# Autodesk Inventor assembly: RearWheelNoLogo
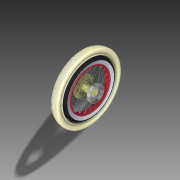
[picture p0: Inventor's stored thumbnail of the model, 180x180]
Saved by Autodesk Inventor 2016 (Build 200138000, 138)
## iProperties
Shininess: 20.0
Length Units: 11269
Angle Units: 11279
Time Units: 11290
Mass Units: 11286
Length Display Precision: 3
Angle Display Precision: 2
Compacted: True
Created: 2001-05-25
Part Number: RearWheelNoLogo
Document SubType Name: Assembly
Designer: Administrator
Density: 0.0
Volumn: 0.0
Area: 0.0
PropertySet Name: Model Information
Control State: 0
Master: False
Checked Out: False
Author: Administrator
## iProperties of the stored document Disk Brake Rotor 230mm.ipt
Created: 2009-08-30
Part Number: Disk Brake Rotor 230mm
Material: SolidWorks Materials|Chrome Stainless Steel|7
Document SubType Name: Modeling
Designer: Yann
Density: 7.8 g/cm^3
Appearance: 229,229,229
Sending System: SolidWorks 2009
Last Author: Administrateur
Last Saved: 2010-11-28
Author: Yann
## Documents named in this file (10)
- **C:\Users\Yann\Documents\GitHub\BIKAIR_CAD\Source\Front_Train\Wheel_spokes\Wheel_spokes.iam*LocalDocs*xCgsrsr1eFgdoe3oxKhlmmklgKg*Disk Brake Rotor 230mm.ipt
- C:\Users\Yann\Documents\GitHub\BIKAIR_CAD\Source\Front_Train\Wheel_spokes\Wheel_spokes.iam
- C:\Users\Yann\Documents\GitHub\BIKAIR_CAD\Source\Front_Train\Wheel_spokes\RearHub.ipt
- C:\Users\Yann\Documents\GitHub\BIKAIR_CAD\Source\Front_Train\Wheel_spokes\ClincherRim2.ipt
- C:\Users\Yann\Documents\GitHub\BIKAIR_CAD\Source\Front_Train\Wheel_spokes\SpokeRear.ipt
- C:\Users\Yann\Documents\GitHub\BIKAIR_CAD\Source\Front_Train\Wheel_spokes\FrontTire.ipt
- C:\Users\Yann\Documents\GitHub\BIKAIR_CAD\Source\Front_Train\Wheel_spokes\RearSprocket.ipt
- C:\Users\Yann\Documents\GitHub\BIKAIR_CAD\Source\Front_Train\Wheel_spokes\BrakeDrum.ipt
- C:\Users\Yann\Documents\GitHub\BIKAIR_CAD\Source\Front_Train\Wheel_spokes\wheel_tyre.ipt
- C:\Users\Yann\Documents\GitHub\BIKAIR_CAD\Source\Front_Train\Wheel_spokes\Disk Brake Rotor 230mm.SLDPRT
## Components (47 placed, 8 different names)
1. RearHub:1 — Mate:1, Mate:2, Mate:3, Mate:5, Mate:7, Mate:9, Mate:11, Insert:1, Insert:2
2. ClincherRim2:1 — Mate:1, Mate:3, Mate:4, Mate:6, Mate:8, Mate:10, Mate:12
3. FrontTire:1 — Mate:11, Mate:12
4. RearSprocket:1 — Insert:1
5. BrakeDrum:1 — Insert:2
6. wheel_tyre:1 — Mate:13, Mate:14
7. Disk Brake Rotor 230mm:1 — Mate:15
8. SpokeRear:1 — Mate:2, Mate:4
9. SpokeRear:2 — Mate:5, Mate:6
10. SpokeRear:3 — Mate:7, Mate:8
11. SpokeRear:4 — Mate:9, Mate:10
12. SpokeRear:5
13. SpokeRear:6
14. SpokeRear:7
15. SpokeRear:8
16. SpokeRear:9
17. SpokeRear:10
18. SpokeRear:11
19. SpokeRear:12
20. SpokeRear:13
21. SpokeRear:14
22. SpokeRear:15
23. SpokeRear:16
24. SpokeRear:17
25. SpokeRear:18
26. SpokeRear:19
27. SpokeRear:20
28. SpokeRear:21
29. SpokeRear:22
30. SpokeRear:23
31. SpokeRear:24
32. SpokeRear:25
33. SpokeRear:26
34. SpokeRear:27
35. SpokeRear:28
36. SpokeRear:29
37. SpokeRear:30
38. SpokeRear:31
39. SpokeRear:32
40. SpokeRear:33
41. SpokeRear:34
42. SpokeRear:35
43. SpokeRear:36
44. SpokeRear:37
45. SpokeRear:38
46. SpokeRear:39
47. SpokeRear:40
## Component patterns: (10 elements, first: SpokeRear:1 + SpokeRear:2 + SpokeRear:3 + SpokeRear:4)
## Relationships (17: Mate 15, Insert 2)
- Mate:1: RearHub:1 ↔ ClincherRim2:1
- Mate:2: RearHub:1 ↔ SpokeRear:1
- Mate:3: RearHub:1 ↔ ClincherRim2:1
- Mate:4: ClincherRim2:1 ↔ SpokeRear:1
- Mate:5: RearHub:1 ↔ SpokeRear:2
- Mate:6: ClincherRim2:1 ↔ SpokeRear:2
- Mate:7: RearHub:1 ↔ SpokeRear:3
- Mate:8: ClincherRim2:1 ↔ SpokeRear:3
- Mate:9: RearHub:1 ↔ SpokeRear:4
- Mate:10: ClincherRim2:1 ↔ SpokeRear:4
- Mate:11: RearHub:1 ↔ FrontTire:1
- Mate:12: ClincherRim2:1 ↔ FrontTire:1
- Insert:1: RearHub:1 ↔ RearSprocket:1
- Insert:2: RearHub:1 ↔ BrakeDrum:1
- Mate:13: wheel_tyre:1
- Mate:14: wheel_tyre:1
- Mate:15: Disk Brake Rotor 230mm:1
